# Autodesk Inventor assembly: Termo
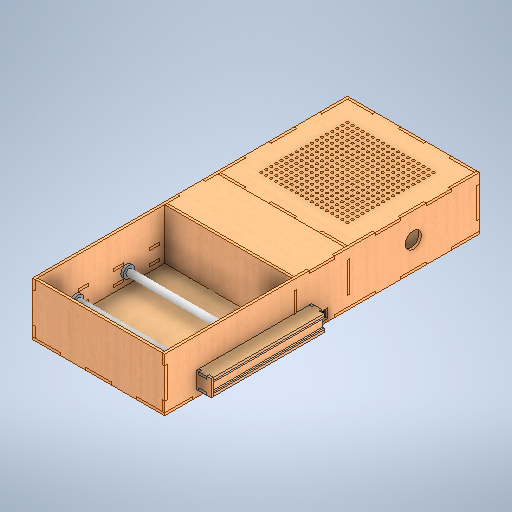
[picture p0: Inventor's stored thumbnail of the model, 512x512]
Saved by Autodesk Inventor 2025 (Build 290162000, 162)
## iProperties
Created: 2024-11-02
Part Number: Termo
Document SubType Name: Assembly
Designer: g.marin
Author: g.marin
## Documents named in this file (16)
- C:\Users\g.marin\Documents\Termoformadora\Termo.iam
- C:\Users\g.marin\Documents\Termoformadora\Base.ipt
- C:\Users\g.marin\Documents\Termoformadora\Lat1.ipt
- C:\Users\g.marin\Documents\Termoformadora\Lat2.ipt
- C:\Users\g.marin\Documents\Termoformadora\Lat3.ipt
- C:\Users\g.marin\Documents\Termoformadora\Lat1(2).ipt
- C:\Users\g.marin\Documents\Termoformadora\Tapa1.ipt
- C:\Users\g.marin\Documents\Termoformadora\Tapa2.ipt
- C:\Users\g.marin\Documents\Termoformadora\Metal1.ipt
- C:\Users\g.marin\Documents\Termoformadora\Metal2.ipt
- C:\Users\g.marin\Documents\Termoformadora\Resistencia.ipt
- C:\Users\g.marin\Documents\Termoformadora\Manija1.ipt
- C:\Users\g.marin\Documents\Termoformadora\Manija2.ipt
- C:\Users\g.marin\Documents\Termoformadora\Manija3.ipt
- C:\Users\g.marin\Documents\Termoformadora\Soporte1.ipt
- C:\Users\g.marin\Documents\Termoformadora\TapaLateral.ipt
## Components (27 placed, 15 different names)
1. Base:1 — Flush:1, Flush:2, Flush:3, Flush:11, Mate:7, Mate:12
2. Lat1:1 — Flush:1, Flush:2, Flush:3, Flush:10, Mate:4, Flush:12, Flush:13, Mate:5, Flush:26
3. Lat2:1 — Flush:10, Mate:4, Flush:11, Mate:6, Flush:17, Flush:18, Flush:20, Flush:21, Flush:24, Mate:13, Flush:27, Mate:15, Mate:16, Mate:17, Mate:18, Mate:19, Mate:20, Flush:28, Mate:21, Mate:22, Mate:23, Flush:29, Mate:24, Flush:30, Flush:33, Mate:25
4. Lat3:1 — Flush:12, Flush:13, Mate:5, Flush:16, Mate:10, Mate:14, Mate:36, Flush:35, Mate:37, Mate:38, Flush:36, Mate:39, Flush:37, Flush:39
5. Lat1(2):1 — Flush:14, Flush:15, Flush:16, Mate:7
6. Lat1(2):2 — Flush:14, Flush:15, Mate:6, Flush:17, Flush:19, Mate:8
7. Tapa1:1 — Flush:18, Flush:19, Mate:8
8. Tapa2:1 — Flush:20, Flush:21, Mate:14
9. Metal1:1 — Flush:25, Mate:11
10. Metal2:1 — Mate:10, Flush:24, Flush:25, Flush:26, Mate:11
11. Lat1:2 — Mate:12, Mate:13, Flush:27
12. Resistencia:1 — Mate:15, Mate:16, Mate:17
13. Resistencia:2 — Mate:18, Mate:19, Mate:20
14. Manija1:1 — Flush:28, Mate:21, Mate:22, Mate:27, Mate:29
15. Manija1:2 — Mate:23, Flush:29, Mate:24, Flush:31, Flush:32, Mate:26, Flush:34, Mate:31, Mate:34
16. Manija2:1 — Flush:30, Flush:31, Flush:32, Mate:28, Mate:30, Mate:35
17. Manija3:1 — Flush:33, Mate:25, Mate:26
18. Soporte1:1 — Flush:34, Mate:30, Mate:31
19. Soporte1:2 — Mate:27, Mate:28, Mate:29, Mate:33
20. TapaLateral:1 — Mate:33, Mate:34, Mate:35
21. Manija1:3 — Mate:36, Flush:35, Mate:37, Flush:38, Mate:40, Mate:41, Flush:40, Flush:42, Mate:44, Mate:47
22. Manija1:4 — Mate:38, Flush:36, Mate:39, Mate:42, Flush:41
23. Manija2:2 — Flush:37, Flush:38, Mate:40, Mate:43, Mate:45, Mate:48
24. Manija3:2 — Flush:39, Mate:41, Flush:40
25. Soporte1:3 — Flush:42, Mate:44, Mate:45
26. Soporte1:4 — Mate:42, Flush:41, Mate:43, Mate:46
27. TapaLateral:2 — Mate:46, Mate:47, Mate:48
## Relationships (77: Mate 43, Flush 34)
- Flush:1: Base:1 ↔ Lat1:1
- Flush:2: Base:1 ↔ Lat1:1
- Flush:3: Base:1 ↔ Lat1:1
- Flush:10: Lat1:1 ↔ Lat2:1
- Mate:4: Lat1:1 ↔ Lat2:1
- Flush:11: Base:1 ↔ Lat2:1
- Flush:12: Lat1:1 ↔ Lat3:1
- Flush:13: Lat1:1 ↔ Lat3:1
- Mate:5: Lat1:1 ↔ Lat3:1
- Flush:14: Lat1(2):1 ↔ Lat1(2):2
- Flush:15: Lat1(2):1 ↔ Lat1(2):2
- Flush:16: Lat3:1 ↔ Lat1(2):1
- Mate:6: Lat2:1 ↔ Lat1(2):2
- Flush:17: Lat2:1 ↔ Lat1(2):2
- Mate:7: Base:1 ↔ Lat1(2):1
- Flush:18: Lat2:1 ↔ Tapa1:1
- Flush:19: Lat1(2):2 ↔ Tapa1:1
- Mate:8: Lat1(2):2 ↔ Tapa1:1
- Flush:20: Lat2:1 ↔ Tapa2:1
- Flush:21: Lat2:1 ↔ Tapa2:1
- Mate:10: Lat3:1 ↔ Metal2:1
- Flush:24: Lat2:1 ↔ Metal2:1
- Flush:25: Metal1:1 ↔ Metal2:1
- Flush:26: Lat1:1 ↔ Metal2:1
- Mate:11: Metal1:1 ↔ Metal2:1
- Mate:12: Base:1 ↔ Lat1:2
- Mate:13: Lat2:1 ↔ Lat1:2
- Flush:27: Lat2:1 ↔ Lat1:2
- Mate:14: Lat3:1 ↔ Tapa2:1
- Mate:15: Lat2:1 ↔ Resistencia:1
- Mate:16: Lat2:1 ↔ Resistencia:1
- Mate:17: Lat2:1 ↔ Resistencia:1
- Mate:18: Lat2:1 ↔ Resistencia:2
- Mate:19: Lat2:1 ↔ Resistencia:2
- Mate:20: Lat2:1 ↔ Resistencia:2
- Flush:28: Lat2:1 ↔ Manija1:1
- Mate:21: Lat2:1 ↔ Manija1:1
- Mate:22: Lat2:1 ↔ Manija1:1
- Mate:23: Lat2:1 ↔ Manija1:2
- Flush:29: Lat2:1 ↔ Manija1:2
- Mate:24: Lat2:1 ↔ Manija1:2
- Flush:30: Lat2:1 ↔ Manija2:1
- Flush:31: Manija1:2 ↔ Manija2:1
- Flush:32: Manija1:2 ↔ Manija2:1
- Flush:33: Lat2:1 ↔ Manija3:1
- Mate:25: Lat2:1 ↔ Manija3:1
- Mate:26: Manija1:2 ↔ Manija3:1
- Mate:27: Manija1:1 ↔ Soporte1:2
- Mate:28: Manija2:1 ↔ Soporte1:2
- Mate:29: Manija1:1 ↔ Soporte1:2
- Flush:34: Manija1:2 ↔ Soporte1:1
- Mate:30: Manija2:1 ↔ Soporte1:1
- Mate:31: Manija1:2 ↔ Soporte1:1
- Mate:33: Soporte1:2 ↔ TapaLateral:1
- Mate:34: Manija1:2 ↔ TapaLateral:1
- Mate:35: Manija2:1 ↔ TapaLateral:1
- Mate:36: Lat3:1 ↔ Manija1:3
- Flush:35: Lat3:1 ↔ Manija1:3
- Mate:37: Lat3:1 ↔ Manija1:3
- Mate:38: Lat3:1 ↔ Manija1:4
- Flush:36: Lat3:1 ↔ Manija1:4
- Mate:39: Lat3:1 ↔ Manija1:4
- Flush:37: Lat3:1 ↔ Manija2:2
- Flush:38: Manija1:3 ↔ Manija2:2
- Mate:40: Manija1:3 ↔ Manija2:2
- Flush:39: Lat3:1 ↔ Manija3:2
- Mate:41: Manija1:3 ↔ Manija3:2
- Flush:40: Manija1:3 ↔ Manija3:2
- Mate:42: Manija1:4 ↔ Soporte1:4
- Flush:41: Manija1:4 ↔ Soporte1:4
- Mate:43: Manija2:2 ↔ Soporte1:4
- Flush:42: Manija1:3 ↔ Soporte1:3
- Mate:44: Manija1:3 ↔ Soporte1:3
- Mate:45: Manija2:2 ↔ Soporte1:3
- Mate:46: Soporte1:4 ↔ TapaLateral:2
- Mate:47: Manija1:3 ↔ TapaLateral:2
- Mate:48: Manija2:2 ↔ TapaLateral:2
